# Autodesk Inventor assembly: Storage Assembly
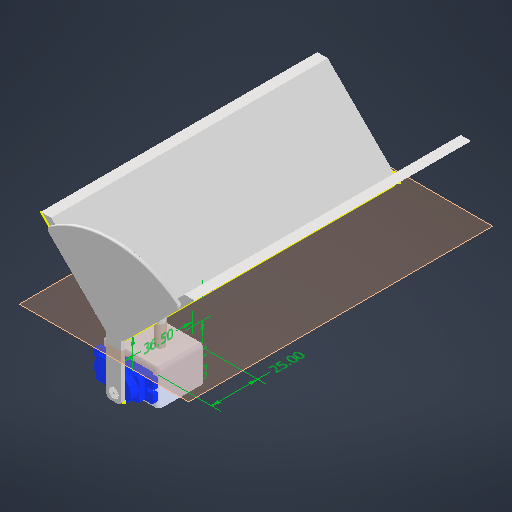
[picture p0: Inventor's stored thumbnail of the model, 512x512]
Saved by Autodesk Inventor 2026.2 (Build 302298010, 298A)
## iProperties
Created: 2026-04-14
Part Number: Storage Assembly
Document SubType Name: Assembly
Designer: lenovo
Author: lenovo
## Documents named in this file (5)
- C:\Users\moham\Desktop\storage\Storage Assembly.iam
- C:\Users\moham\Desktop\storage\Part2.ipt
- C:\Users\moham\Desktop\storage\Part1#2 .ipt
- C:\Users\moham\Desktop\storage\Servo housing.ipt
- C:\Users\moham\Desktop\storage\Part1_sG90.ipt
## Components (4 placed, 4 different names)
1. Part2:1
2. Part1#2 :1 — Mate:4
3. Servo housing:1 — Mate:1, Mate:2, Mate:3
4. Part1_sG90:1 — Mate:1, Mate:2, Mate:3, Mate:4
## Relationships (4: Mate 4)
- Mate:1: Servo housing:1 ↔ Part1_sG90:1
- Mate:2: Servo housing:1 ↔ Part1_sG90:1
- Mate:3: Servo housing:1 ↔ Part1_sG90:1
- Mate:4: Part1#2 :1 ↔ Part1_sG90:1
